# Autodesk Inventor assembly: Anglerfish_v1
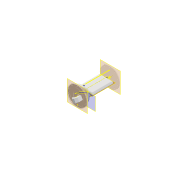
[picture p0: Inventor's stored thumbnail of the model, 180x180]
Saved by Autodesk Inventor 2022 (Build 260153000, 153)
## iProperties
Created: 2022-04-02
Part Number: Anglerfish_v1
Document SubType Name: Assembly
Designer: Prakash Lab
Author: Prakash Lab
## Documents named in this file (9)
- C:\Users\PrakashLab\Documents\Matchboxscope\INVENTOR\Anglerfish_v1.iam
- C:\Users\PrakashLab\Documents\Matchboxscope\INVENTOR\Matchboxscope_middle2_v1.ipt
- C:\Users\PrakashLab\Documents\Matchboxscope\INVENTOR\Matchboxscope_Lightperiscope_V0.ipt
- C:\Users\PrakashLab\Documents\Matchboxscope\INVENTOR\Matchboxscope_bottom_v0.ipt
- C:\Users\PrakashLab\Documents\Matchboxscope\INVENTOR\00_ESP3-CAM.iam
- C:\Users\PrakashLab\Documents\Matchboxscope\INVENTOR\Matchboxscope_lenstube_v0.ipt
- C:\Users\PrakashLab\Documents\Matchboxscope\INVENTOR\00_Powerbank.ipt
- C:\Users\PrakashLab\Documents\Matchboxscope\INVENTOR\Anglerfish_Tube_v0.ipt
- C:\Users\PrakashLab\Documents\Matchboxscope\INVENTOR\Anglerfish_Frontwindow_v0.ipt
## Components (9 placed, 8 different names)
1. Matchboxscope_middle2_v1:1 — Insert:1, Angle:1, Mate:5
2. Matchboxscope_Lightperiscope_V0:1
3. Matchboxscope_bottom_v0:1 — Mate:1, Mate:2, Mate:3, Mate:4, Flush:1, Mate:5, Mate:6, Mate:7, Mate:8, Mate:9, Flush:5
4. 00_ESP3-CAM:1 [sub-assembly] — Mate:4, Flush:1, Insert:1
5. Matchboxscope_lenstube_v0:1
6. 00_Powerbank:1 — Mate:7, Mate:8, Mate:9, Flush:4, Flush:6
7. Anglerfish_Tube_v0:1 — Mate:6, Angle:2, Flush:2, Flush:3, Flush:4, Insert:2, Flush:5, Flush:6
8. Anglerfish_Frontwindow_v0:1 — Flush:2, Flush:3
9. Anglerfish_Frontwindow_v0:2 — Insert:2
## Relationships (19: Mate 9, Flush 6, Insert 2, Angle 2)
- Mate:1: Matchboxscope_bottom_v0:1
- Mate:2: Matchboxscope_bottom_v0:1
- Mate:3: Matchboxscope_bottom_v0:1
- Mate:4: Matchboxscope_bottom_v0:1 ↔ 00_ESP3-CAM:1
- Flush:1: Matchboxscope_bottom_v0:1 ↔ 00_ESP3-CAM:1
- Insert:1: Matchboxscope_middle2_v1:1 ↔ 00_ESP3-CAM:1
- Angle:1 (0 deg): Matchboxscope_middle2_v1:1
- Mate:5: Matchboxscope_middle2_v1:1 ↔ Matchboxscope_bottom_v0:1
- Mate:6: Matchboxscope_bottom_v0:1 ↔ Anglerfish_Tube_v0:1
- Angle:2 (0 deg): Anglerfish_Tube_v0:1
- Mate:7: Matchboxscope_bottom_v0:1 ↔ 00_Powerbank:1
- Mate:8: Matchboxscope_bottom_v0:1 ↔ 00_Powerbank:1
- Mate:9 (5 mm): Matchboxscope_bottom_v0:1 ↔ 00_Powerbank:1
- Flush:2: Anglerfish_Tube_v0:1 ↔ Anglerfish_Frontwindow_v0:1
- Flush:3: Anglerfish_Tube_v0:1 ↔ Anglerfish_Frontwindow_v0:1
- Flush:4: 00_Powerbank:1 ↔ Anglerfish_Tube_v0:1
- Insert:2: Anglerfish_Tube_v0:1 ↔ Anglerfish_Frontwindow_v0:2
- Flush:5: Matchboxscope_bottom_v0:1 ↔ Anglerfish_Tube_v0:1
- Flush:6: 00_Powerbank:1 ↔ Anglerfish_Tube_v0:1
